# Autodesk Inventor assembly: SCST8-10
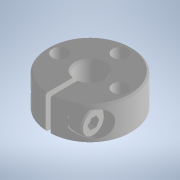
[picture p0: Inventor's stored thumbnail of the model, 180x180]
Saved by Autodesk Inventor 2021 (Build 250183000, 183)
## iProperties
Category: PARTsolutions
Company: MISUMI
Created: 2025-08-06
Part Number: SCST8-10
Catalog Web Link: www.cadenas.de
Description: SCST, PSCST, SSCST, SCSTR, PSCSTR, SSCSTR-Set Collars - Slit 3 Hole/3 Tap - Standard Type -
Vendor: MISUMI
Document SubType Name: Assembly
Designer: psAdmin
Manufacturer: MISUMI
Mass: 3.73216 g
Surface Area: 28.0062 cm^2
Volume: 3.73216 cm^3
Density: 1 g/cm^3
Title: SCST8-10
Author: Cadenas PARTsolutions
Comments: Set Collars - Slit 3 Hole/3 Tap - Standard Type -
PSOL_IDENT_0: {$CADENAS_DATA/23d-libs/misumi/metric/03_set_collars/scst_asmtab.prj},219 {VTYP=3D},{STYP=ASSTAB},{N
PSOL_IDENT_1: B=SCST8-10},{LINA=SCST8-10},{NN=SCST, PSCST, SSCST, SCSTR, PSCSTR, SSCSTR},{DATE=29.11.2024 04:05:21
PSOL_IDENT_2: },{GEOMDATE=15.09.2021 06:07:55},{VERSION=},{LINEID=50},{WBVAR=TS,MAT,ST,BS},{WBNUMERIC=BS}  {NB=SCS
PSOL_IDENT_3: T8-10},{LINA=SCST8-10},{KT=DUMMY},{PN=SCST8-10},{TYPE=SCST},{TS=3H},{TSALG= '3H' , '3-Hole' , '3T' ,
PSOL_IDENT_4: '3-Tapped' },{MAT=S45C},{ST=BO},{STALG= 'BO' , 'Black Oxide' , 'ENP' , 'Electroless Nickel Plating'
PSOL_IDENT_5: },{AC=Hex Socket Head Cap Screw 1 pc.},{ACMAT=4137 Alloy Steel},{D=8},{BS=10},{BALG= 8 , 10 , 15 },
PSOL_IDENT_6: {D1=25},{M=M4},{M3D=4},{DD=4.5},{R=3.75},{W=1.5},{X=8.0},{Y=5},{P=18},{C=0.5},{S=4.5},{M1=-},{M13D=0
PSOL_IDENT_7: },{L=12},{PPATH=scst/scst_templ.prj}
NB: SCST8-10
NN: SCST, PSCST, SSCST, SCSTR, PSCSTR, SSCSTR
NT: Set Collars - Slit 3 Hole/3 Tap - Standard Type -
NBSYN: $PN.
LINA: SCST8-10
CATALOG: Misumi
PN: SCST8-10
TS: 3-Hole
MAT: 1045 Carbon Steel
ST: Black Oxide
AC: Hex Socket Head Cap Screw 1 pc.
ACMAT: 4137 Alloy Steel
D: 8
BS: 10
D1: 25
M: M4
DD: 4.5
R: 3.75
W: 1.5
X: 8
Y: 5
P: 18
C: 0.5
S: 4.5
M1: -
SUPPLIER: MISUMI
ARTICLENO: SCST8-10
BOMINFO: SCST8-10
CREATOR: CADENAS GmbH
## Documents named in this file (3)
- e:\temp\worker_COMMON_55\temp\tmp_3980_14_Pmjqb\format_0\SCST8-10.iam
- e:\temp\worker_COMMON_55\temp\tmp_3980_14_Pmjqb\format_0\SCST8-10b.ipt
- e:\temp\worker_COMMON_55\temp\tmp_3980_14_Pmjqb\format_0\BOLT4-12.ipt
## Components (2 placed, 2 different names)
1. SCST8-10b:1 — to_bolt_XY@1 <-> to_cp_XY@2, to_bolt_Z@1 <-> to_cp_Z@2, to_bolt_YZ@1 <-> to_cp_YZ@2
2. BOLT4-12:1 — to_bolt_XY@1 <-> to_cp_XY@2, to_bolt_Z@1 <-> to_cp_Z@2, to_bolt_YZ@1 <-> to_cp_YZ@2
## Relationships (3: Mate 2, Angle 1)
- to_bolt_XY@1 <-> to_cp_XY@2 [Mate]: SCST8-10b:1 ↔ BOLT4-12:1
- to_bolt_Z@1 <-> to_cp_Z@2 [Mate]: SCST8-10b:1 ↔ BOLT4-12:1
- to_bolt_YZ@1 <-> to_cp_YZ@2 [Angle] (0 deg): SCST8-10b:1 ↔ BOLT4-12:1
